# Autodesk Inventor assembly: chumacera de 20 mm
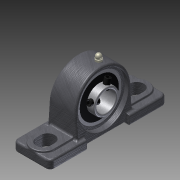
[picture p0: Inventor's stored thumbnail of the model, 180x180]
Saved by Autodesk Inventor 2012 (Build 160160000, 160)
## iProperties
Created: 2012-06-13
Part Number: chumacera de 20 mm
Document SubType Name: Assembly
Designer: Luis
Author: Luis
## Documents named in this file (6)
- J:\Gravity2012\Imported Components\Chumacera 34\chumacera de 20 mm.iam
- J:\Gravity2012\Imported Components\Chumacera 34\1.ipt
- J:\Gravity2012\Imported Components\Chumacera 34\2.ipt
- J:\Gravity2012\Imported Components\Chumacera 34\3.ipt
- J:\Gravity2012\Imported Components\Chumacera 34\4.ipt
- J:\Gravity2012\Imported Components\Chumacera 34\5.ipt
## Components (6 placed, 5 different names)
1. 1:1 — Insert:1, Mate:3
2. 2:1 — Insert:1, Insert:2, Mate:1, Mate:2
3. 3:1 — Insert:2
4. 4:1 — Mate:2
5. 4:2 — Mate:1
6. 5:1 — Mate:3
## Relationships (5: Mate 3, Insert 2)
- Insert:1: 1:1 ↔ 2:1
- Insert:2: 2:1 ↔ 3:1
- Mate:1: 2:1 ↔ 4:2
- Mate:2: 2:1 ↔ 4:1
- Mate:3: 1:1 ↔ 5:1
